# Autodesk Inventor assembly: Overview
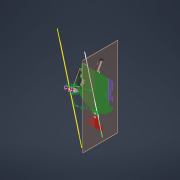
[picture p0: Inventor's stored thumbnail of the model, 180x180]
Saved by Autodesk Inventor 2022 (Build 260153000, 153)
## iProperties
Created: 2021-10-05
Part Number: Overview
Document SubType Name: Assembly
Designer: shiok
Mass: 71.5322 g
Surface Area: 774.809 cm^2
Volume: 60.689 cm^3
Density: 1.17867 g/cm^3
Author: shiok
## Documents named in this file (8)
- C:\Users\shiok\Documents\GitHub\murakumo\inventor\Overview.iam
- C:\Users\shiok\Documents\GitHub\murakumo\inventor\flame.ipt
- C:\Users\shiok\Documents\GitHub\murakumo\inventor\sensor.ipt
- C:\Users\shiok\Documents\GitHub\murakumo\inventor\SideSensorCircuit.ipt
- C:\Users\shiok\Documents\GitHub\murakumo\inventor\top.ipt
- C:\Users\shiok\Documents\GitHub\murakumo\inventor\jump.ipt
- C:\Users\shiok\Documents\GitHub\murakumo\inventor\SideSensorMount.ipt
- C:\Users\shiok\Documents\GitHub\murakumo\inventor\Motor.iam
## Components (7 placed, 7 different names)
1. flame:1 — フラッシュ:1, フラッシュ:2, フラッシュ:3, メイト:15, フラッシュ:7, メイト:16, メイト:23, メイト:24, メイト:25, メイト:30
2. sensor:1 — フラッシュ:6, メイト:15, フラッシュ:7, メイト:17, メイト:18
3. top:1 — メイト:26, メイト:27, メイト:28
4. jump:1 — メイト:16, メイト:17, メイト:18
5. SideSensorCircuit:1 — メイト:19, フラッシュ:8, 挿入:22, 挿入:23
6. SideSensorMount:1 — メイト:19, フラッシュ:8, 挿入:22, 挿入:23, メイト:29, メイト:30
7. Motor:1 [sub-assembly] — メイト:23, メイト:24, メイト:25, メイト:26, メイト:27, メイト:28, メイト:29
## Relationships (21: Mate 13, Flush 6, Insert 2)
- フラッシュ:1 [Flush]: flame:1
- フラッシュ:2 [Flush]: flame:1
- フラッシュ:3 [Flush]: flame:1
- フラッシュ:6 [Flush]: sensor:1
- メイト:15 [Mate]: flame:1 ↔ sensor:1
- フラッシュ:7 [Flush]: flame:1 ↔ sensor:1
- メイト:16 [Mate]: flame:1 ↔ jump:1
- メイト:17 [Mate]: sensor:1 ↔ jump:1
- メイト:18 [Mate]: sensor:1 ↔ jump:1
- メイト:19 [Mate]: SideSensorCircuit:1 ↔ SideSensorMount:1
- フラッシュ:8 [Flush]: SideSensorCircuit:1 ↔ SideSensorMount:1
- 挿入:22 [Insert]: SideSensorCircuit:1 ↔ SideSensorMount:1
- 挿入:23 [Insert]: SideSensorCircuit:1 ↔ SideSensorMount:1
- メイト:23 [Mate]: flame:1 ↔ Motor:1
- メイト:24 [Mate]: flame:1 ↔ Motor:1
- メイト:25 [Mate]: flame:1 ↔ Motor:1
- メイト:26 [Mate]: top:1 ↔ Motor:1
- メイト:27 [Mate]: top:1 ↔ Motor:1
- メイト:28 [Mate]: top:1 ↔ Motor:1
- メイト:29 [Mate]: SideSensorMount:1 ↔ Motor:1
- メイト:30 [Mate]: flame:1 ↔ SideSensorMount:1
